# Autodesk Inventor assembly: Magnet_MIR
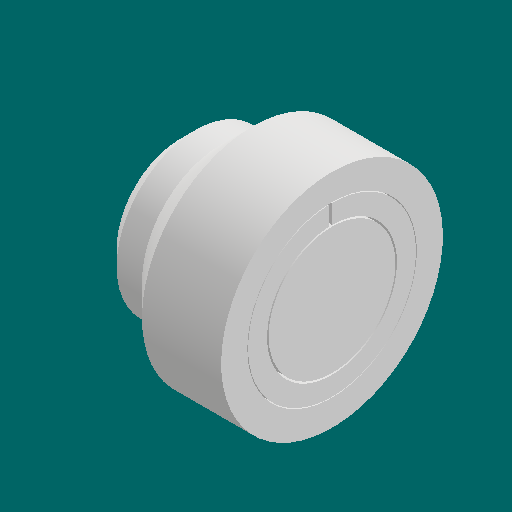
[picture p0: Inventor's stored thumbnail of the model, 512x512]
Saved by Autodesk Inventor 2023 (Build 270158000, 158)
## iProperties
Created: 2022-03-29
Part Number: Magnet_MIR
Document SubType Name: Assembly
Designer: hide
Author: neko2
## Documents named in this file (4)
- C:\Users\hide\Desktop\SaponseEx\CAD\mirror\Magnet_MIR.iam
- C:\Users\hide\Desktop\SaponseEx\CAD\mirror\Magnet_MIR.ipt
- C:\Users\hide\Desktop\SaponseEx\CAD\mirror\Spacer_MIR.ipt
- C:\Users\hide\Desktop\SaponseEx\CAD\mirror\MagnetMounter_MIR.ipt
## Components (3 placed, 3 different names)
1. Magnet_MIR:1 — フラッシュ:1, メイト:2
2. Spacer_MIR:1 — フラッシュ:1, メイト:2, フラッシュ:2, メイト:1
3. MagnetMounter_MIR:1 — フラッシュ:2, メイト:1
## Relationships (4: Flush 2, Mate 2)
- フラッシュ:1 [Flush]: Magnet_MIR:1 ↔ Spacer_MIR:1
- メイト:2 [Mate]: Magnet_MIR:1 ↔ Spacer_MIR:1
- フラッシュ:2 [Flush]: Spacer_MIR:1 ↔ MagnetMounter_MIR:1
- メイト:1 [Mate]: Spacer_MIR:1 ↔ MagnetMounter_MIR:1
